# Autodesk Inventor assembly: Bot 1
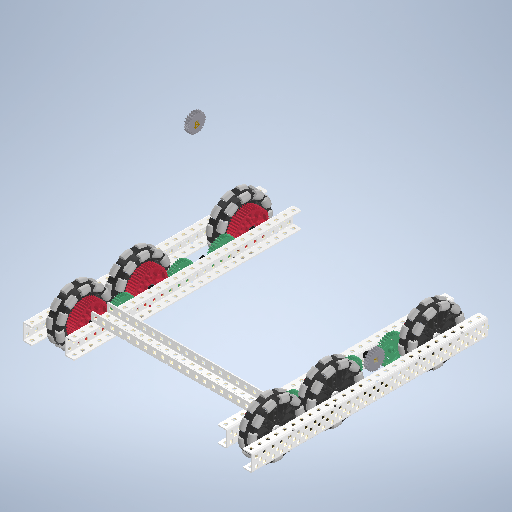
[picture p0: Inventor's stored thumbnail of the model, 512x512]
Saved by Autodesk Inventor 2025.2 (Build 292293000, 293)
## iProperties
Created: 2025-03-17
Part Number: Bot 1
Document SubType Name: Assembly
Designer: Jahan
Author: Jahan
## Documents named in this file (18)
- C:\1629X-7700R-Worlds-Bot\Bot 1\Bot 1.iam
- C:\1629X-7700R-Worlds-Bot\VEX-CAD-Inventor-1.4.2\Structure\C Channel\Aluminum 1x2x1\Alu C 1x2x1x27.ipt
- C:\1629X-7700R-Worlds-Bot\VEX-CAD-Inventor-1.4.2\Structure\C Channel\Aluminum 1x2x1\Alu C 1x2x1x19.ipt
- C:\1629X-7700R-Worlds-Bot\VEX-CAD-Inventor-1.4.2\Structure\C Channel\Aluminum 1x2x1\Alu C 1x2x1x28.ipt
- C:\1629X-7700R-Worlds-Bot\VEX-CAD-Inventor-1.4.2\Motion\Gears\HS Gear.iam
- C:\1629X-7700R-Worlds-Bot\VEX-CAD-Inventor-1.4.2\Motion\Wheels\Omni Wheel\3.25 Omni AS, No Insert.iam
- C:\1629X-7700R-Worlds-Bot\VEX-CAD-Inventor-1.4.2\Motion\Wheels\Omni Wheel.iam
- C:\1629X-7700R-Worlds-Bot\VEX-CAD-Inventor-1.4.2\Motion\Gears\HS Gear\HS 48T Gear, Circle.iam
- C:\1629X-7700R-Worlds-Bot\VEX-CAD-Inventor-1.4.2\Structure\Standoff.ipt
- C:\1629X-7700R-Worlds-Bot\VEX-CAD-Inventor-1.4.2\Structure\Standoff\Standoff .50.ipt
- C:\1629X-7700R-Worlds-Bot\VEX-CAD-Inventor-1.4.2\Motion\Spacers\Washer Teflon.ipt
- C:\1629X-7700R-Worlds-Bot\VEX-CAD-Inventor-1.4.2\Motion\Spacers\Spacer Nylon .375 OD\NSpacer .375 OD x .125.ipt
- C:\1629X-7700R-Worlds-Bot\VEX-CAD-Inventor-1.4.2\Motion\Spacers\Spacer Nylon .375 OD.ipt
- C:\1629X-7700R-Worlds-Bot\VEX-CAD-Inventor-1.4.2\Motion\Spacers\Washer Teflon\TWasher .375 OD x .06250.ipt
- C:\1629X-7700R-Worlds-Bot\VEX-CAD-Inventor-1.4.2\Structure\Hardware\alu_nylock.ipt
- C:\1629X-7700R-Worlds-Bot\VEX-CAD-Inventor-1.4.2\Motion\Gears\LS 36T Gear.ipt
- C:\1629X-7700R-Worlds-Bot\VEX-CAD-Inventor-1.4.2\Motion\Gears\HS Gear\24T HS Gear Cut.iam
- C:\1629X-7700R-Worlds-Bot\VEX-CAD-Inventor-1.4.2\Motion\Shaft LS\Bearing Flat Low Profile.ipt
## Components (54 placed, 12 different names)
1. Alu C 1x2x1x19:1 — Insert:1, Insert:2, Insert:3, Insert:4
2. Alu C 1x2x1x27:1 — Insert:3, Insert:4, Insert:19, Insert:32, Insert:40, Insert:41
3. Alu C 1x2x1x27:2 — Insert:1, Insert:2, Insert:5, Insert:6, Insert:59, Insert:66, Insert:67, Insert:69
4. Alu C 1x2x1x27:3 — Insert:5, Insert:6, Insert:7, Insert:8, Insert:9, Insert:10
5. Alu C 1x2x1x28:1 — Insert:7, Insert:8, Insert:52, Insert:58, Insert:65
6. Alu C 1x2x1x28:2 — Insert:9, Insert:10, Insert:25, Insert:31, Insert:39, Insert:43, Insert:44, Insert:45, Insert:46
7. LS 36T Gear:1 — Insert:19
8. HS 48T Gear, Circle:3 [sub-assembly] — Mate:1
9. 3.25 Omni AS, No Insert:4 [sub-assembly] — Mate:1
10. NSpacer .375 OD x .125:2
11. TWasher .375 OD x .06250:2 — Insert:23
12. alu_nylock:3 — Insert:23, Insert:24
13. Standoff .50:3 — Insert:24, Insert:25
14. HS 48T Gear, Circle:4 [sub-assembly] — Mate:2
15. 3.25 Omni AS, No Insert:5 [sub-assembly] — Mate:2
16. NSpacer .375 OD x .125:3
17. TWasher .375 OD x .06250:3
18. alu_nylock:4
19. Standoff .50:4 — Insert:31
20. LS 36T Gear:2 — Insert:32
21. HS 48T Gear, Circle:5 [sub-assembly] — Mate:3
22. 3.25 Omni AS, No Insert:6 [sub-assembly] — Mate:3
23. NSpacer .375 OD x .125:4
24. TWasher .375 OD x .06250:4
25. alu_nylock:5
26. Standoff .50:5 — Insert:39
27. LS 36T Gear:4 — Insert:40
28. 24T HS Gear Cut:2 [sub-assembly] — Insert:42
29. NSpacer .375 OD x .125:5 — Insert:41, Insert:42
30. Bearing Flat Low Profile:1 — Insert:43, Insert:44
31. Bearing Flat Low Profile:2 — Insert:45, Insert:46
32. HS 48T Gear, Circle:6 [sub-assembly]
33. 3.25 Omni AS, No Insert:7 [sub-assembly]
34. NSpacer .375 OD x .125:6
35. TWasher .375 OD x .06250:5
36. alu_nylock:6
37. Standoff .50:6 — Insert:52
38. HS 48T Gear, Circle:7 [sub-assembly]
39. 3.25 Omni AS, No Insert:8 [sub-assembly]
40. NSpacer .375 OD x .125:7
41. TWasher .375 OD x .06250:6
42. alu_nylock:7
43. Standoff .50:7 — Insert:58
44. LS 36T Gear:5 — Insert:59
45. HS 48T Gear, Circle:8 [sub-assembly]
46. 3.25 Omni AS, No Insert:9 [sub-assembly]
47. NSpacer .375 OD x .125:8
48. TWasher .375 OD x .06250:7
49. alu_nylock:8
50. Standoff .50:8 — Insert:65
51. LS 36T Gear:6 — Insert:66
52. LS 36T Gear:7 — Insert:67
53. NSpacer .375 OD x .125:9 — Insert:69
54. 24T HS Gear Cut:4 [sub-assembly]
## Relationships (65: Insert 59, Mate 6)
- Insert:1: Alu C 1x2x1x19:1 ↔ Alu C 1x2x1x27:2
- Insert:2: Alu C 1x2x1x19:1 ↔ Alu C 1x2x1x27:2
- Insert:3: Alu C 1x2x1x19:1 ↔ Alu C 1x2x1x27:1
- Insert:4: Alu C 1x2x1x19:1 ↔ Alu C 1x2x1x27:1
- Insert:5: Alu C 1x2x1x27:2 ↔ Alu C 1x2x1x27:3
- Insert:6: Alu C 1x2x1x27:2 ↔ Alu C 1x2x1x27:3
- Insert:7: Alu C 1x2x1x27:3 ↔ Alu C 1x2x1x28:1
- Insert:8: Alu C 1x2x1x27:3 ↔ Alu C 1x2x1x28:1
- Insert:9: Alu C 1x2x1x27:3 ↔ Alu C 1x2x1x28:2
- Insert:10: Alu C 1x2x1x27:3 ↔ Alu C 1x2x1x28:2
- Insert:19: Alu C 1x2x1x27:1 ↔ LS 36T Gear:1
- [Insert]: HS 48T Gear, Circle:3 ↔ 3.25 Omni AS, No Insert:4
- [Insert]: HS 48T Gear, Circle:3 ↔ NSpacer .375 OD x .125:2
- [Insert]: 3.25 Omni AS, No Insert:4 ↔ TWasher .375 OD x .06250:2
- Insert:23: TWasher .375 OD x .06250:2 ↔ alu_nylock:3
- Insert:24: alu_nylock:3 ↔ Standoff .50:3
- Insert:25: Alu C 1x2x1x28:2 ↔ Standoff .50:3
- [Insert]: HS 48T Gear, Circle:4 ↔ 3.25 Omni AS, No Insert:5
- [Insert]: HS 48T Gear, Circle:4 ↔ NSpacer .375 OD x .125:3
- [Insert]: 3.25 Omni AS, No Insert:5 ↔ TWasher .375 OD x .06250:3
- [Insert]: TWasher .375 OD x .06250:3 ↔ alu_nylock:4
- [Insert]: alu_nylock:4 ↔ Standoff .50:4
- Insert:31: Alu C 1x2x1x28:2 ↔ Standoff .50:4
- Insert:32: Alu C 1x2x1x27:1 ↔ LS 36T Gear:2
- [Insert]: HS 48T Gear, Circle:5 ↔ 3.25 Omni AS, No Insert:6
- [Insert]: HS 48T Gear, Circle:5 ↔ NSpacer .375 OD x .125:4
- [Insert]: 3.25 Omni AS, No Insert:6 ↔ TWasher .375 OD x .06250:4
- [Insert]: TWasher .375 OD x .06250:4 ↔ alu_nylock:5
- [Insert]: alu_nylock:5 ↔ Standoff .50:5
- Insert:39: Alu C 1x2x1x28:2 ↔ Standoff .50:5
- Insert:40: Alu C 1x2x1x27:1 ↔ LS 36T Gear:4
- Mate:1: HS 48T Gear, Circle:3 ↔ 3.25 Omni AS, No Insert:4
- Mate:2: HS 48T Gear, Circle:4 ↔ 3.25 Omni AS, No Insert:5
- Mate:3: HS 48T Gear, Circle:5 ↔ 3.25 Omni AS, No Insert:6
- Insert:41: Alu C 1x2x1x27:1 ↔ NSpacer .375 OD x .125:5
- Insert:42: 24T HS Gear Cut:2 ↔ NSpacer .375 OD x .125:5
- Insert:43: Alu C 1x2x1x28:2 ↔ Bearing Flat Low Profile:1
- Insert:44: Alu C 1x2x1x28:2 ↔ Bearing Flat Low Profile:1
- Insert:45: Alu C 1x2x1x28:2 ↔ Bearing Flat Low Profile:2
- Insert:46: Alu C 1x2x1x28:2 ↔ Bearing Flat Low Profile:2
- [Insert]: HS 48T Gear, Circle:6 ↔ 3.25 Omni AS, No Insert:7
- [Insert]: HS 48T Gear, Circle:6 ↔ NSpacer .375 OD x .125:6
- [Insert]: 3.25 Omni AS, No Insert:7 ↔ TWasher .375 OD x .06250:5
- [Insert]: TWasher .375 OD x .06250:5 ↔ alu_nylock:6
- [Insert]: alu_nylock:6 ↔ Standoff .50:6
- [Mate]: HS 48T Gear, Circle:6 ↔ 3.25 Omni AS, No Insert:7
- Insert:52: Alu C 1x2x1x28:1 ↔ Standoff .50:6
- [Insert]: HS 48T Gear, Circle:7 ↔ 3.25 Omni AS, No Insert:8
- [Insert]: HS 48T Gear, Circle:7 ↔ NSpacer .375 OD x .125:7
- [Insert]: 3.25 Omni AS, No Insert:8 ↔ TWasher .375 OD x .06250:6
- [Insert]: TWasher .375 OD x .06250:6 ↔ alu_nylock:7
- [Insert]: alu_nylock:7 ↔ Standoff .50:7
- [Mate]: HS 48T Gear, Circle:7 ↔ 3.25 Omni AS, No Insert:8
- Insert:58: Alu C 1x2x1x28:1 ↔ Standoff .50:7
- Insert:59: Alu C 1x2x1x27:2 ↔ LS 36T Gear:5
- [Insert]: HS 48T Gear, Circle:8 ↔ 3.25 Omni AS, No Insert:9
- [Insert]: HS 48T Gear, Circle:8 ↔ NSpacer .375 OD x .125:8
- [Insert]: 3.25 Omni AS, No Insert:9 ↔ TWasher .375 OD x .06250:7
- [Insert]: TWasher .375 OD x .06250:7 ↔ alu_nylock:8
- [Insert]: alu_nylock:8 ↔ Standoff .50:8
- [Mate]: HS 48T Gear, Circle:8 ↔ 3.25 Omni AS, No Insert:9
- Insert:65: Alu C 1x2x1x28:1 ↔ Standoff .50:8
- Insert:66: Alu C 1x2x1x27:2 ↔ LS 36T Gear:6
- Insert:67: Alu C 1x2x1x27:2 ↔ LS 36T Gear:7
- Insert:69: Alu C 1x2x1x27:2 ↔ NSpacer .375 OD x .125:9
## Named parameters: d122_d116 = 0 mm, d123_d117 = 0 mm, d124_d119 = 0 mm, d129_d122_d116 = 0 mm, d130_d123_d117 = 0 mm, d131_d124_d119 = 0 mm, d132_d126 = 0 mm, d133_d127 = 0 mm, d144_d129_d122_d116 = 0 mm, d145_d130_d123_d117 = 0 mm, d146_d131_d124_d119 = 0 mm, d147_d132_d126 = 0 mm, d148_d133_d127 = 0 mm, d162_d127 = 0 mm, d163_d153 = 0 mm, d164_d122_d116 = 0 mm, d165_d123_d117 = 0 mm, d166_d124_d119 = 0 mm, d167_d126 = 0 mm, d169_d127 = 0 mm, d170_d153 = 0 mm, d171_d122_d116 = 0 mm, d172_d123_d117 = 0 mm, d173_d124_d119 = 0 mm, d174_d126 = 0 mm, d177_d169_d127 = 0 mm, d178_d170_d153 = 0 mm, d179_d171_d122_d116 = 0 mm, d180_d172_d123_d117 = 0 mm, d181_d173_d124_d119 = 0 mm, d182_d174_d126 = 0 mm
